# Autodesk Inventor assembly: CyberOrto
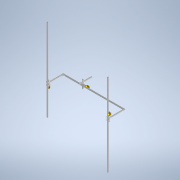
[picture p0: Inventor's stored thumbnail of the model, 180x180]
Saved by Autodesk Inventor 2022 (Build 260153000, 153)
## iProperties
RuleStatus: InUse
Created: 2021-12-29
Part Number: CyberOrto
Document SubType Name: Assembly
Designer: matte
Author: matte
## Documents named in this file (29)
- C:\Users\matte\Documents\GitHub\MDM-CyberOrto-CAD\CyberOrto.iam
- C:\Users\matte\Documents\GitHub\MDM-CyberOrto-CAD\Pezzi singoli\Trave Principale.ipt
- C:\Users\matte\Documents\GitHub\MDM-CyberOrto-CAD\Pezzi singoli\Supporto SX.ipt
- C:\Users\matte\Documents\GitHub\MDM-CyberOrto-CAD\Parker components\03-Brackets_Gussets_Plates\09-Machined Gussets\20-102.ipt
- C:\Users\matte\Documents\GitHub\MDM-CyberOrto-CAD\Parker components\02-Fasteners\10-Standard T-Nuts\20-050.ipt
- C:\Users\matte\Documents\GitHub\MDM-CyberOrto-CAD\Parker components\02-Fasteners\16-Screws\01-Metric Screws\01-Button Head\24-118-8.ipt
- C:\Users\matte\Documents\GitHub\MDM-CyberOrto-CAD\Guida a terra.iam
- C:\Users\matte\Documents\GitHub\MDM-CyberOrto-CAD\Parker components\05-Handles_Hinges\13-Pivot Joints\23-010.iam
- C:\Users\matte\Documents\GitHub\MDM-CyberOrto-CAD\Parker components\02-Fasteners\10-Standard T-Nuts\20-058.ipt
- C:\Users\matte\Documents\GitHub\MDM-CyberOrto-CAD\Parker components\02-Fasteners\16-Screws\01-Metric Screws\01-Button Head\24-116-8.ipt
- C:\Users\matte\Documents\GitHub\MDM-CyberOrto-CAD\Pezzi singoli\Supporto DX.ipt
- C:\Users\matte\Documents\GitHub\MDM-CyberOrto-CAD\Parker components\02-Fasteners\16-Screws\01-Metric Screws\01-Button Head\24-120-8.ipt
- C:\Users\matte\Documents\GitHub\MDM-CyberOrto-CAD\Pezzi singoli\Supporto lineare\Carrello semplice.iam
- C:\Users\matte\Documents\GitHub\MDM-CyberOrto-CAD\Platform.ipt
- C:\Users\matte\Documents\GitHub\MDM-CyberOrto-CAD\Parker components\02-Fasteners\16-Screws\01-Metric Screws\01-Button Head\24-130-6.ipt
- C:\Users\matte\Documents\GitHub\MDM-CyberOrto-CAD\Parker components\02-Fasteners\15-T-Bolts_Nuts_Washers\03-Washers\24-700-6.ipt
- C:\Users\matte\Documents\GitHub\MDM-CyberOrto-CAD\Parker components\02-Fasteners\15-T-Bolts_Nuts_Washers\02-Nuts\24-706-6.ipt
- C:\Users\matte\Documents\GitHub\MDM-CyberOrto-CAD\Servo Motor 50W\bch2mba531ca5c.ipt
- C:\Users\matte\Documents\GitHub\MDM-CyberOrto-CAD\Rack_Pinion\Rack gear scaled1.ipt
- C:\Users\matte\Documents\GitHub\MDM-CyberOrto-CAD\Rack_Pinion\pinion_scaled1.ipt
- C:\Users\matte\Documents\GitHub\MDM-CyberOrto-CAD\Inventor Support\Content Center Files\it-IT\ISO 1580\ISO 1580 - M4 x 12_.ipt
- C:\Users\matte\Documents\GitHub\MDM-CyberOrto-CAD\Inventor Support\Content Center Files\it-IT\AS 1474(1)\AS 1474 - M4(1).ipt
- C:\Users\matte\Documents\GitHub\MDM-CyberOrto-CAD\Trave a terra\Trave a terra.iam
- C:\Users\matte\Documents\GitHub\MDM-CyberOrto-CAD\Racks.iam
- C:\Users\matte\Documents\GitHub\MDM-CyberOrto-CAD\Parker components\02-Fasteners\16-Screws\01-Metric Screws\03-Socket Head\24-320-8SS.ipt
- C:\Users\matte\Documents\GitHub\MDM-CyberOrto-CAD\Parker components\02-Fasteners\10-Standard T-Nuts\20-058SS.ipt
- C:\Users\matte\Documents\GitHub\MDM-CyberOrto-CAD\Torretta.iam
- C:\Users\matte\Documents\GitHub\MDM-CyberOrto-CAD\Pezzi singoli\13-106_f.ipt
- C:\Users\matte\Documents\GitHub\MDM-CyberOrto-CAD\Pezzi singoli\13-513.ipt
## Components (129 placed, 28 different names)
1. Trave Principale:1 — Coincidente:1, Coincidente:2, Coincidente:3, Allineato:1, Coincidente:4, Allineato:2, Coincidente:5, Coincidente:10, Coincidente:40, Allineato:5, Allineato:6, Coincidente:41, Angolo:1, Angolo:7, Allineato:119, Coincidente:238, Allineato:120, Coincidente:239, Coincidente:245, Coincidente:257, Angolo:9, Allineato:141, Coincidente:259, Coincidente:260, Allineato:142, Coincidente:261, Coincidente:262, Allineato:143, Allineato:144, Coincidente:265
2. Supporto SX:1 — Allineato:1, Coincidente:4, Allineato:2, Coincidente:6, Allineato:3, Coincidente:7, Coincidente:15, Coincidente:16, Coincidente:23, Coincidente:28, Coincidente:29, Coincidente:30
3. Supporto DX:1 — Coincidente:45, Allineato:7, Allineato:8, Coincidente:48, Allineato:9, Allineato:10
4. Torretta:1 [sub-assembly] — Angolo:7, Coincidente:258, Coincidente:265, Allineato:145
5. pinion_scaled1:3 — Coincidente:258, Allineato:146
6. 13-106_f:1 — Allineato:142, Coincidente:261, Coincidente:262, Coincidente:264, Allineato:145
7. 13-106_f:2 — Allineato:141, Coincidente:259, Coincidente:260, Coincidente:263
8. 13-513:1 — Allineato:143, Coincidente:264
9. 13-513:2 — Allineato:144, Coincidente:263
10. 24-118-8:3 — Coincidente:19, Coincidente:20
11. 24-118-8:4 — Coincidente:21, Coincidente:22
12. 20-050:2 — Coincidente:10, Coincidente:11, Coincidente:12
13. 24-118-8:1 — Coincidente:13, Coincidente:14
14. 24-118-8:2 — Coincidente:17, Coincidente:18
15. 20-102:1 — Coincidente:5, Coincidente:6, Allineato:3, Coincidente:8, Coincidente:9, Coincidente:11, Coincidente:12, Coincidente:13, Coincidente:14, Coincidente:17, Coincidente:18, Coincidente:19, Coincidente:20, Coincidente:21, Coincidente:22
16. 20-050:1 — Coincidente:7, Coincidente:8, Coincidente:9
17. 24-118-8:5 — Coincidente:31, Coincidente:32, Coincidente:33
18. 24-118-8:6 — Coincidente:34, Coincidente:35
19. 24-118-8:7 — Coincidente:38, Coincidente:39
20. 24-118-8:8 — Coincidente:36, Coincidente:37
21. Guida a terra:1 [sub-assembly] — Coincidente:15, Coincidente:16, Coincidente:23, Coincidente:32, Coincidente:33, Coincidente:34, Coincidente:35, Coincidente:36, Coincidente:37, Coincidente:38, Coincidente:39, Coincidente:138, Coincidente:139, Allineato:61, Coincidente:141, Coincidente:143, Coincidente:145, Coincidente:162, Coincidente:210, Allineato:115
22. 20-050:3 — Coincidente:27, Allineato:4, Coincidente:28, Coincidente:30, Coincidente:31
23. 20-050:4 — Coincidente:27, Allineato:4, Coincidente:29
24. 23-010:1 [sub-assembly] — Coincidente:40, Allineato:5, Allineato:6, Coincidente:43, Coincidente:44, Coincidente:45, Allineato:7, Allineato:8, Coincidente:46, Coincidente:47
25. 20-058:1 — Coincidente:41, Angolo:1, Coincidente:42
26. 24-116-8:1 — Coincidente:42, Coincidente:43, Coincidente:44
27. 24-120-8:1 — Coincidente:46, Coincidente:47
28. 24-120-8:2 — Coincidente:51, Coincidente:52
29. Carrello semplice:1 [sub-assembly] — Coincidente:48, Allineato:9, Allineato:10, Coincidente:51, Coincidente:52, Coincidente:53, Allineato:13, Coincidente:54, Coincidente:56, Coincidente:58, Coincidente:60, Coincidente:62, Angolo:2, Angolo:3, Angolo:4, Allineato:59, Coincidente:130
30. 24-130-6:1 — Inserimento:1, Coincidente:61
31. 24-700-6:1 — Inserimento:1, Inserimento:7
32. 24-706-6:1 — Coincidente:55, Coincidente:56
33. 24-130-6:2 — Coincidente:59
34. 24-700-6:3 — Inserimento:6
35. 24-130-6:3 — Coincidente:57
36. 24-700-6:2 — Inserimento:8
37. 24-130-6:4 — Coincidente:55
38. 24-700-6:4 — Inserimento:5
39. 24-706-6:2 — Coincidente:57, Coincidente:58
40. 24-706-6:3 — Coincidente:61, Coincidente:62
41. 24-706-6:4 — Coincidente:59, Coincidente:60
42. Platform:1 — Coincidente:53, Allineato:13, Coincidente:54, Inserimento:5, Inserimento:6, Inserimento:7, Inserimento:8, Coincidente:66, Coincidente:67, Coincidente:68, Coincidente:114, Coincidente:117, Coincidente:121, Coincidente:125, Coincidente:129
43. ISO 1580 M4 x 12:2 — Coincidente:126, Coincidente:127, Coincidente:128
44. AS 1474 - Metrico M4:2 — Coincidente:120, Coincidente:121
45. AS 1474 - Metrico M4:3 — Coincidente:124, Coincidente:125
46. AS 1474 - Metrico M4:4 — Coincidente:128, Coincidente:129
47. ISO 1580 M4 x 12:4 — Coincidente:118, Coincidente:119, Coincidente:120
48. ISO 1580 M4 x 12:3 — Coincidente:122, Coincidente:123, Coincidente:124
49. AS 1474 - Metrico M4:1 — Coincidente:116, Coincidente:117
50. ISO 1580 M4 x 12:1 — Coincidente:114, Coincidente:115, Coincidente:116
51. bch2mba531ca5c:1 — Coincidente:66, Coincidente:67, Coincidente:68, Coincidente:113, Coincidente:115, Coincidente:118, Coincidente:119, Coincidente:122, Coincidente:123, Coincidente:126, Coincidente:127
52. 24-706-6:8 — Coincidente:142, Coincidente:143
53. 24-706-6:7 — Coincidente:140, Coincidente:141
54. 24-706-6:6 — Coincidente:144, Coincidente:145
55. 24-700-6:8
56. 24-130-6:8 — Coincidente:146
57. 24-700-6:7
58. 24-130-6:7 — Coincidente:144
59. 24-700-6:6
60. 24-706-6:5 — Coincidente:146, Coincidente:162
61. 24-700-6:5
62. Platform:3 — Coincidente:138, Coincidente:139, Allineato:61, Coincidente:158, Coincidente:159, Coincidente:160, Coincidente:164, Coincidente:166, Coincidente:167, Coincidente:168
63. 24-130-6:5 — Coincidente:142
64. 24-130-6:6 — Coincidente:140
65. bch2mba531ca5c:2 — Coincidente:158, Coincidente:161, Coincidente:211
66. ISO 1580 M4 x 12:5 — Coincidente:161
67. AS 1474 - Metrico M4:5 — Coincidente:167
68. ISO 1580 M4 x 12:6 — Coincidente:159, Coincidente:163
69. AS 1474 - Metrico M4:6 — Coincidente:168
70. AS 1474 - Metrico M4:7 — Coincidente:165, Coincidente:166
71. ISO 1580 M4 x 12:7 — Coincidente:165
72. AS 1474 - Metrico M4:8 — Coincidente:163, Coincidente:164
73. ISO 1580 M4 x 12:8 — Coincidente:160
74. pinion_scaled1:1 — Coincidente:113, Allineato:87
75. Trave a terra:1 [sub-assembly] — Angolo:2, Angolo:3, Angolo:4, Allineato:59, Coincidente:130, Coincidente:169, Angolo:5, Coincidente:171, Allineato:62, Allineato:88, Coincidente:187, Coincidente:189
76. 20-058SS:2 — Coincidente:188, Coincidente:189
77. 20-058SS:1 — Coincidente:186, Coincidente:187
78. Racks:5 [sub-assembly] — Allineato:73, Allineato:74, Coincidente:177, Allineato:75, Allineato:76, Coincidente:178
79. Racks:6 [sub-assembly] — Allineato:75, Allineato:76, Coincidente:178, Coincidente:180, Allineato:77, Allineato:78
80. Racks:7 [sub-assembly] — Coincidente:180, Allineato:77, Allineato:78, Allineato:79, Allineato:80, Coincidente:181
81. Racks:8 [sub-assembly] — Allineato:79, Allineato:80, Coincidente:181, Coincidente:182, Allineato:81, Allineato:82
82. Racks:9 [sub-assembly] — Coincidente:182, Allineato:81, Allineato:82, Allineato:85, Allineato:86, Coincidente:185
83. Rack gear scaled1:2 — Allineato:85, Allineato:86, Coincidente:185
84. 24-320-8SS:3
85. 24-320-8SS:4 — Coincidente:188
86. Racks:4 [sub-assembly] — Coincidente:174, Allineato:67, Allineato:68, Allineato:69, Allineato:70, Coincidente:175
87. Racks:3 [sub-assembly] — Allineato:71, Coincidente:176, Allineato:72, Allineato:73, Allineato:74, Coincidente:177
88. Racks:2 [sub-assembly] — Allineato:69, Allineato:70, Coincidente:175, Allineato:71, Coincidente:176, Allineato:72
89. Rack gear scaled1:1 — Coincidente:170, Coincidente:171, Allineato:62, Allineato:63, Allineato:64, Coincidente:172, Allineato:65, Coincidente:173, Allineato:66
90. 24-320-8SS:1 — Coincidente:172, Allineato:65, Coincidente:186
91. 24-320-8SS:2 — Coincidente:173, Allineato:66
92. Racks:1 [sub-assembly] — Coincidente:169, Angolo:5, Coincidente:170, Allineato:63, Allineato:64, Coincidente:174, Allineato:67, Allineato:68, Allineato:87, Allineato:88
93. pinion_scaled1:2 — Coincidente:211, Allineato:116
94. Trave a terra:2 [sub-assembly] — Coincidente:210, Allineato:115
95. 20-058SS:4
96. 24-320-8SS:8
97. 24-320-8SS:7
98. Rack gear scaled1:4
99. Racks:18 [sub-assembly]
100. Racks:17 [sub-assembly]
101. Racks:16 [sub-assembly]
102. Racks:15 [sub-assembly]
103. Racks:14 [sub-assembly]
104. Racks:11 [sub-assembly] — Allineato:116
105. Racks:12 [sub-assembly]
106. Racks:13 [sub-assembly]
107. Racks:10 [sub-assembly]
108. Rack gear scaled1:3
109. 24-320-8SS:5
110. 24-320-8SS:6
111. 20-058SS:3
112. Rack gear scaled1:5 — Allineato:119, Coincidente:238, Allineato:120, Angolo:8, Coincidente:246, Allineato:131
113. 24-320-8SS:9
114. 24-320-8SS:10
115. 20-058SS:5 — Angolo:8, Coincidente:239
116. Racks:19 [sub-assembly] — Coincidente:250, Allineato:139, Allineato:140
117. Racks:20 [sub-assembly]
118. Racks:21 [sub-assembly] — Coincidente:245
119. Racks:22 [sub-assembly]
120. Racks:23 [sub-assembly] — Allineato:146
121. Racks:24 [sub-assembly] — Coincidente:246, Allineato:131
122. Rack gear scaled1:6 — Coincidente:250, Allineato:134, Allineato:137, Coincidente:255, Allineato:138, Allineato:139, Allineato:140
123. 24-320-8SS:11 — Coincidente:251
124. 24-320-8SS:12
125. 20-050:5 — Coincidente:251, Allineato:134, Coincidente:254
126. Rack gear scaled1:7 — Allineato:137, Coincidente:255, Allineato:138
127. 24-320-8SS:14 — Coincidente:254
128. 24-320-8SS:13 — Coincidente:256
129. 20-058SS:6 — Coincidente:256, Coincidente:257, Angolo:9
## Relationships (302: Mate 179, Flush 98, Insert 16, Angle 9)
- Coincidente:1 [Mate]: Trave Principale:1
- Coincidente:2 [Mate]: Trave Principale:1
- Coincidente:3 [Mate]: Trave Principale:1
- Allineato:1 [Flush]: Trave Principale:1 ↔ Supporto SX:1
- Coincidente:4 [Mate]: Trave Principale:1 ↔ Supporto SX:1
- Allineato:2 [Flush]: Trave Principale:1 ↔ Supporto SX:1
- Coincidente:5 [Mate]: Trave Principale:1 ↔ 20-102:1
- Coincidente:6 [Mate]: Supporto SX:1 ↔ 20-102:1
- Allineato:3 [Flush]: Supporto SX:1 ↔ 20-102:1
- Coincidente:7 [Mate]: Supporto SX:1 ↔ 20-050:1
- Coincidente:8 [Mate]: 20-102:1 ↔ 20-050:1
- Coincidente:9 [Mate]: 20-102:1 ↔ 20-050:1
- Coincidente:10 [Mate]: Trave Principale:1 ↔ 20-050:2
- Coincidente:11 [Mate]: 20-050:2 ↔ 20-102:1
- Coincidente:12 [Mate]: 20-050:2 ↔ 20-102:1
- Coincidente:13 [Mate]: 24-118-8:1 ↔ 20-102:1
- Coincidente:14 [Mate]: 24-118-8:1 ↔ 20-102:1
- Coincidente:15 [Mate]: Supporto SX:1 ↔ Guida a terra:1
- Coincidente:16 [Mate]: Supporto SX:1 ↔ Guida a terra:1
- Coincidente:17 [Mate]: 24-118-8:2 ↔ 20-102:1
- Coincidente:18 [Mate]: 24-118-8:2 ↔ 20-102:1
- Coincidente:19 [Mate]: 24-118-8:3 ↔ 20-102:1
- Coincidente:20 [Mate]: 24-118-8:3 ↔ 20-102:1
- Coincidente:21 [Mate]: 24-118-8:4 ↔ 20-102:1
- Coincidente:22 [Mate]: 24-118-8:4 ↔ 20-102:1
- Coincidente:23 [Mate]: Supporto SX:1 ↔ Guida a terra:1
- Coincidente:27 [Mate]: 20-050:3 ↔ 20-050:4
- Allineato:4 [Flush]: 20-050:3 ↔ 20-050:4
- Coincidente:28 [Mate]: Supporto SX:1 ↔ 20-050:3
- Coincidente:29 [Mate]: Supporto SX:1 ↔ 20-050:4
- Coincidente:30 [Mate]: Supporto SX:1 ↔ 20-050:3
- Coincidente:31 [Mate]: 24-118-8:5 ↔ 20-050:3
- Coincidente:32 [Mate]: 24-118-8:5 ↔ Guida a terra:1
- Coincidente:33 [Mate]: 24-118-8:5 ↔ Guida a terra:1
- Coincidente:34 [Mate]: 24-118-8:6 ↔ Guida a terra:1
- Coincidente:35 [Mate]: 24-118-8:6 ↔ Guida a terra:1
- Coincidente:36 [Mate]: 24-118-8:8 ↔ Guida a terra:1
- Coincidente:37 [Mate]: 24-118-8:8 ↔ Guida a terra:1
- Coincidente:38 [Mate]: 24-118-8:7 ↔ Guida a terra:1
- Coincidente:39 [Mate]: 24-118-8:7 ↔ Guida a terra:1
- Coincidente:40 [Mate]: Trave Principale:1 ↔ 23-010:1
- Allineato:5 [Flush]: Trave Principale:1 ↔ 23-010:1
- Allineato:6 [Flush]: Trave Principale:1 ↔ 23-010:1
- Coincidente:41 [Mate]: Trave Principale:1 ↔ 20-058:1
- Angolo:1 [Angle] (0 deg): Trave Principale:1 ↔ 20-058:1
- Coincidente:42 [Mate]: 20-058:1 ↔ 24-116-8:1
- Coincidente:43 [Mate]: 23-010:1 ↔ 24-116-8:1
- Coincidente:44 [Mate]: 23-010:1 ↔ 24-116-8:1
- Coincidente:45 [Mate]: Supporto DX:1 ↔ 23-010:1
- Allineato:7 [Flush]: Supporto DX:1 ↔ 23-010:1
- Allineato:8 [Flush]: Supporto DX:1 ↔ 23-010:1
- Coincidente:46 [Mate]: 23-010:1 ↔ 24-120-8:1
- Coincidente:47 [Mate]: 23-010:1 ↔ 24-120-8:1
- Coincidente:48 [Mate]: Supporto DX:1 ↔ Carrello semplice:1
- Allineato:9 [Flush]: Supporto DX:1 ↔ Carrello semplice:1
- Allineato:10 [Flush]: Supporto DX:1 ↔ Carrello semplice:1
- Coincidente:51 [Mate]: 24-120-8:2 ↔ Carrello semplice:1
- Coincidente:52 [Mate]: 24-120-8:2 ↔ Carrello semplice:1
- Coincidente:53 [Mate]: Carrello semplice:1 ↔ Platform:1
- Allineato:13 [Flush]: Carrello semplice:1 ↔ Platform:1
- Coincidente:54 [Mate]: Carrello semplice:1 ↔ Platform:1
- Inserimento:1: 24-130-6:1 ↔ 24-700-6:1
- [Insert]: 24-130-6:2 ↔ 24-700-6:2
- [Insert]: 24-700-6:3 ↔ 24-130-6:3
- [Insert]: 24-130-6:4 ↔ 24-700-6:4
- Inserimento:5: 24-700-6:4 ↔ Platform:1
- Inserimento:6: 24-700-6:3 ↔ Platform:1
- Inserimento:7: 24-700-6:1 ↔ Platform:1
- Inserimento:8: 24-700-6:2 ↔ Platform:1
- Coincidente:55 [Mate]: 24-706-6:1 ↔ 24-130-6:4
- Coincidente:56 [Mate]: Carrello semplice:1 ↔ 24-706-6:1
- Coincidente:57 [Mate]: 24-130-6:3 ↔ 24-706-6:2
- Coincidente:58 [Mate]: Carrello semplice:1 ↔ 24-706-6:2
- Coincidente:59 [Mate]: 24-130-6:2 ↔ 24-706-6:4
- Coincidente:60 [Mate]: Carrello semplice:1 ↔ 24-706-6:4
- Coincidente:61 [Mate]: 24-130-6:1 ↔ 24-706-6:3
- Coincidente:62 [Mate]: Carrello semplice:1 ↔ 24-706-6:3
- Coincidente:66 [Mate]: Platform:1 ↔ bch2mba531ca5c:1
- Coincidente:67 [Mate]: Platform:1 ↔ bch2mba531ca5c:1
- Coincidente:68 [Mate]: Platform:1 ↔ bch2mba531ca5c:1
- Coincidente:113 [Mate]: bch2mba531ca5c:1 ↔ pinion_scaled1:1
- Coincidente:114 [Mate]: Platform:1 ↔ ISO 1580 M4 x 12:1
- Coincidente:115 [Mate]: ISO 1580 M4 x 12:1 ↔ bch2mba531ca5c:1
- Coincidente:116 [Mate]: AS 1474 - Metrico M4:1 ↔ ISO 1580 M4 x 12:1
- Coincidente:117 [Mate]: Platform:1 ↔ AS 1474 - Metrico M4:1
- Coincidente:118 [Mate]: ISO 1580 M4 x 12:4 ↔ bch2mba531ca5c:1
- Coincidente:119 [Mate]: ISO 1580 M4 x 12:4 ↔ bch2mba531ca5c:1
- Coincidente:120 [Mate]: AS 1474 - Metrico M4:2 ↔ ISO 1580 M4 x 12:4
- Coincidente:121 [Mate]: Platform:1 ↔ AS 1474 - Metrico M4:2
- Coincidente:122 [Mate]: ISO 1580 M4 x 12:3 ↔ bch2mba531ca5c:1
- Coincidente:123 [Mate]: ISO 1580 M4 x 12:3 ↔ bch2mba531ca5c:1
- Coincidente:124 [Mate]: AS 1474 - Metrico M4:3 ↔ ISO 1580 M4 x 12:3
- Coincidente:125 [Mate]: Platform:1 ↔ AS 1474 - Metrico M4:3
- Coincidente:126 [Mate]: ISO 1580 M4 x 12:2 ↔ bch2mba531ca5c:1
- Coincidente:127 [Mate]: ISO 1580 M4 x 12:2 ↔ bch2mba531ca5c:1
- Coincidente:128 [Mate]: ISO 1580 M4 x 12:2 ↔ AS 1474 - Metrico M4:4
- Coincidente:129 [Mate]: Platform:1 ↔ AS 1474 - Metrico M4:4
- Angolo:2 [Angle] (0 deg): Carrello semplice:1 ↔ Trave a terra:1
- Angolo:3 [Angle] (0 deg): Carrello semplice:1 ↔ Trave a terra:1
- Angolo:4 [Angle] (0 deg): Carrello semplice:1 ↔ Trave a terra:1
- Allineato:59 [Flush] (19 mm): Carrello semplice:1 ↔ Trave a terra:1
- Coincidente:130 [Mate] (20 mm): Carrello semplice:1 ↔ Trave a terra:1
- [Insert]: 24-700-6:5 ↔ 24-130-6:5
- [Insert]: 24-700-6:6 ↔ 24-130-6:6
- [Insert]: 24-700-6:7 ↔ 24-130-6:7
- [Insert]: 24-700-6:8 ↔ 24-130-6:8
- [Insert]: 24-700-6:8 ↔ Platform:3
- [Insert]: 24-700-6:7 ↔ Platform:3
- [Insert]: 24-700-6:5 ↔ Platform:3
- [Insert]: 24-700-6:6 ↔ Platform:3
- Coincidente:138 [Mate]: Guida a terra:1 ↔ Platform:3
- Coincidente:139 [Mate]: Guida a terra:1 ↔ Platform:3
- Allineato:61 [Flush]: Guida a terra:1 ↔ Platform:3
- Coincidente:140 [Mate]: 24-706-6:7 ↔ 24-130-6:6
- Coincidente:141 [Mate]: Guida a terra:1 ↔ 24-706-6:7
- Coincidente:142 [Mate]: 24-706-6:8 ↔ 24-130-6:5
- Coincidente:143 [Mate]: Guida a terra:1 ↔ 24-706-6:8
- Coincidente:144 [Mate]: 24-706-6:6 ↔ 24-130-6:7
- Coincidente:145 [Mate]: Guida a terra:1 ↔ 24-706-6:6
- Coincidente:146 [Mate]: 24-130-6:8 ↔ 24-706-6:5
- [Mate]: bch2mba531ca5c:2 ↔ ISO 1580 M4 x 12:5
- [Mate]: ISO 1580 M4 x 12:5 ↔ AS 1474 - Metrico M4:5
- [Mate]: bch2mba531ca5c:2 ↔ ISO 1580 M4 x 12:8
- [Mate]: bch2mba531ca5c:2 ↔ ISO 1580 M4 x 12:8
- [Mate]: AS 1474 - Metrico M4:6 ↔ ISO 1580 M4 x 12:8
- [Mate]: bch2mba531ca5c:2 ↔ ISO 1580 M4 x 12:7
- [Mate]: bch2mba531ca5c:2 ↔ ISO 1580 M4 x 12:7
- [Mate]: bch2mba531ca5c:2 ↔ ISO 1580 M4 x 12:6
- [Mate]: bch2mba531ca5c:2 ↔ ISO 1580 M4 x 12:6
- Coincidente:158 [Mate]: Platform:3 ↔ bch2mba531ca5c:2
- Coincidente:159 [Mate]: Platform:3 ↔ ISO 1580 M4 x 12:6
- Coincidente:160 [Mate]: Platform:3 ↔ ISO 1580 M4 x 12:8
- Coincidente:161 [Mate]: bch2mba531ca5c:2 ↔ ISO 1580 M4 x 12:5
- Coincidente:162 [Mate]: Guida a terra:1 ↔ 24-706-6:5
- Coincidente:163 [Mate]: ISO 1580 M4 x 12:6 ↔ AS 1474 - Metrico M4:8
- Coincidente:164 [Mate]: Platform:3 ↔ AS 1474 - Metrico M4:8
- Coincidente:165 [Mate]: AS 1474 - Metrico M4:7 ↔ ISO 1580 M4 x 12:7
- Coincidente:166 [Mate]: Platform:3 ↔ AS 1474 - Metrico M4:7
- Coincidente:167 [Mate]: Platform:3 ↔ AS 1474 - Metrico M4:5
- Coincidente:168 [Mate]: Platform:3 ↔ AS 1474 - Metrico M4:6
- Coincidente:169 [Mate]: Trave a terra:1 ↔ Racks:1
- Angolo:5 [Angle] (0 deg): Trave a terra:1 ↔ Racks:1
- Coincidente:170 [Mate]: Rack gear scaled1:1 ↔ Racks:1
- Coincidente:171 [Mate]: Trave a terra:1 ↔ Rack gear scaled1:1
- Allineato:62 [Flush]: Trave a terra:1 ↔ Rack gear scaled1:1
- Allineato:63 [Flush]: Rack gear scaled1:1 ↔ Racks:1
- Allineato:64 [Flush]: Rack gear scaled1:1 ↔ Racks:1
- Coincidente:172 [Mate]: Rack gear scaled1:1 ↔ 24-320-8SS:1
- Allineato:65 [Flush]: Rack gear scaled1:1 ↔ 24-320-8SS:1
- Coincidente:173 [Mate]: Rack gear scaled1:1 ↔ 24-320-8SS:2
- Allineato:66 [Flush]: Rack gear scaled1:1 ↔ 24-320-8SS:2
- Coincidente:174 [Mate]: Racks:4 ↔ Racks:1
- Allineato:67 [Flush]: Racks:4 ↔ Racks:1
- Allineato:68 [Flush]: Racks:4 ↔ Racks:1
- Allineato:69 [Flush]: Racks:4 ↔ Racks:2
- Allineato:70 [Flush]: Racks:4 ↔ Racks:2
- Coincidente:175 [Mate]: Racks:4 ↔ Racks:2
- Allineato:71 [Flush]: Racks:3 ↔ Racks:2
- Coincidente:176 [Mate]: Racks:3 ↔ Racks:2
- Allineato:72 [Flush]: Racks:3 ↔ Racks:2
- Allineato:73 [Flush]: Racks:5 ↔ Racks:3
- Allineato:74 [Flush]: Racks:5 ↔ Racks:3
- Coincidente:177 [Mate]: Racks:5 ↔ Racks:3
- Allineato:75 [Flush]: Racks:5 ↔ Racks:6
- Allineato:76 [Flush]: Racks:5 ↔ Racks:6
- Coincidente:178 [Mate]: Racks:5 ↔ Racks:6
- Coincidente:180 [Mate]: Racks:6 ↔ Racks:7
- Allineato:77 [Flush]: Racks:6 ↔ Racks:7
- Allineato:78 [Flush]: Racks:6 ↔ Racks:7
- Allineato:79 [Flush]: Racks:7 ↔ Racks:8
- Allineato:80 [Flush]: Racks:7 ↔ Racks:8
- Coincidente:181 [Mate]: Racks:7 ↔ Racks:8
- Coincidente:182 [Mate]: Racks:8 ↔ Racks:9
- Allineato:81 [Flush]: Racks:8 ↔ Racks:9
- Allineato:82 [Flush]: Racks:8 ↔ Racks:9
- [Mate]: Rack gear scaled1:2 ↔ 24-320-8SS:3
- [Flush]: Rack gear scaled1:2 ↔ 24-320-8SS:3
- [Mate]: Rack gear scaled1:2 ↔ 24-320-8SS:4
- [Flush]: Rack gear scaled1:2 ↔ 24-320-8SS:4
- Allineato:85 [Flush]: Racks:9 ↔ Rack gear scaled1:2
- Allineato:86 [Flush]: Racks:9 ↔ Rack gear scaled1:2
- Coincidente:185 [Mate]: Racks:9 ↔ Rack gear scaled1:2
- Allineato:87 [Flush]: pinion_scaled1:1 ↔ Racks:1
- Allineato:88 [Flush] (-13 mm): Trave a terra:1 ↔ Racks:1
- Coincidente:186 [Mate]: 20-058SS:1 ↔ 24-320-8SS:1
- Coincidente:187 [Mate]: Trave a terra:1 ↔ 20-058SS:1
- Coincidente:188 [Mate]: 20-058SS:2 ↔ 24-320-8SS:4
- Coincidente:189 [Mate]: Trave a terra:1 ↔ 20-058SS:2
- [Mate]: Trave a terra:2 ↔ Racks:10
- [Angle] (0 deg): Trave a terra:2 ↔ Racks:10
- [Mate]: Racks:10 ↔ Rack gear scaled1:3
- [Mate]: Trave a terra:2 ↔ Rack gear scaled1:3
- [Flush]: Trave a terra:2 ↔ Rack gear scaled1:3
- [Flush]: Racks:10 ↔ Rack gear scaled1:3
- [Flush]: Racks:10 ↔ Rack gear scaled1:3
- [Mate]: Rack gear scaled1:3 ↔ 24-320-8SS:5
- [Flush]: Rack gear scaled1:3 ↔ 24-320-8SS:5
- [Mate]: Rack gear scaled1:3 ↔ 24-320-8SS:6
- [Flush]: Rack gear scaled1:3 ↔ 24-320-8SS:6
- [Mate]: Racks:13 ↔ Racks:10
- [Flush]: Racks:13 ↔ Racks:10
- [Flush]: Racks:13 ↔ Racks:10
- [Flush]: Racks:11 ↔ Racks:13
- [Flush]: Racks:11 ↔ Racks:13
- [Mate]: Racks:11 ↔ Racks:13
- [Flush]: Racks:11 ↔ Racks:12
- [Mate]: Racks:11 ↔ Racks:12
- [Flush]: Racks:11 ↔ Racks:12
- [Flush]: Racks:14 ↔ Racks:12
- [Flush]: Racks:14 ↔ Racks:12
- [Mate]: Racks:14 ↔ Racks:12
- [Flush]: Racks:15 ↔ Racks:14
- [Flush]: Racks:15 ↔ Racks:14
- [Mate]: Racks:15 ↔ Racks:14
- [Mate]: Racks:16 ↔ Racks:15
- [Flush]: Racks:16 ↔ Racks:15
- [Flush]: Racks:16 ↔ Racks:15
- [Flush]: Racks:17 ↔ Racks:16
- [Flush]: Racks:17 ↔ Racks:16
- [Mate]: Racks:17 ↔ Racks:16
- [Mate]: Racks:18 ↔ Racks:17
- [Flush]: Racks:18 ↔ Racks:17
- [Flush]: Racks:18 ↔ Racks:17
- [Mate]: 24-320-8SS:7 ↔ Rack gear scaled1:4
- [Flush]: 24-320-8SS:7 ↔ Rack gear scaled1:4
- [Mate]: 24-320-8SS:8 ↔ Rack gear scaled1:4
- [Flush]: 24-320-8SS:8 ↔ Rack gear scaled1:4
- [Flush]: Rack gear scaled1:4 ↔ Racks:18
- [Flush]: Rack gear scaled1:4 ↔ Racks:18
- [Mate]: Rack gear scaled1:4 ↔ Racks:18
- [Flush] (-13 mm): Trave a terra:2 ↔ Racks:10
- [Mate]: 24-320-8SS:5 ↔ 20-058SS:3
- [Mate]: Trave a terra:2 ↔ 20-058SS:3
- [Mate]: 20-058SS:4 ↔ 24-320-8SS:8
- [Mate]: Trave a terra:2 ↔ 20-058SS:4
- Coincidente:210 [Mate] (20 mm): Guida a terra:1 ↔ Trave a terra:2
- Allineato:115 [Flush] (19 mm): Guida a terra:1 ↔ Trave a terra:2
- Coincidente:211 [Mate]: bch2mba531ca5c:2 ↔ pinion_scaled1:2
- Allineato:116 [Flush]: pinion_scaled1:2 ↔ Racks:11
- Angolo:7 [Angle] (180 deg): Trave Principale:1 ↔ Torretta:1
- [Mate]: Rack gear scaled1:5 ↔ 24-320-8SS:9
- [Flush]: Rack gear scaled1:5 ↔ 24-320-8SS:9
- [Mate]: Rack gear scaled1:5 ↔ 24-320-8SS:10
- [Flush]: Rack gear scaled1:5 ↔ 24-320-8SS:10
- [Mate]: 24-320-8SS:10 ↔ 20-058SS:5
- Allineato:119 [Flush]: Trave Principale:1 ↔ Rack gear scaled1:5
- Coincidente:238 [Mate]: Trave Principale:1 ↔ Rack gear scaled1:5
- Allineato:120 [Flush] (13 mm): Trave Principale:1 ↔ Rack gear scaled1:5
- Angolo:8 [Angle] (0 deg): Rack gear scaled1:5 ↔ 20-058SS:5
- Coincidente:239 [Mate]: Trave Principale:1 ↔ 20-058SS:5
- [Mate]: Racks:19 ↔ Racks:22
- [Flush]: Racks:19 ↔ Racks:22
- [Flush]: Racks:19 ↔ Racks:22
- [Flush]: Racks:20 ↔ Racks:22
- [Flush]: Racks:20 ↔ Racks:22
- [Mate]: Racks:20 ↔ Racks:22
- [Flush]: Racks:20 ↔ Racks:21
- [Mate]: Racks:20 ↔ Racks:21
- [Flush]: Racks:20 ↔ Racks:21
- [Flush]: Racks:21 ↔ Racks:23
- [Flush]: Racks:21 ↔ Racks:23
- [Mate]: Racks:21 ↔ Racks:23
- [Flush]: Racks:23 ↔ Racks:24
- [Flush]: Racks:23 ↔ Racks:24
- [Mate]: Racks:23 ↔ Racks:24
- Coincidente:245 [Mate]: Trave Principale:1 ↔ Racks:21
- Coincidente:246 [Mate]: Rack gear scaled1:5 ↔ Racks:24
- Allineato:131 [Flush]: Rack gear scaled1:5 ↔ Racks:24
- [Mate]: Rack gear scaled1:6 ↔ 24-320-8SS:11
- [Flush]: Rack gear scaled1:6 ↔ 24-320-8SS:11
- [Mate]: Rack gear scaled1:6 ↔ 24-320-8SS:12
- [Flush]: Rack gear scaled1:6 ↔ 24-320-8SS:12
- Coincidente:250 [Mate]: Racks:19 ↔ Rack gear scaled1:6
- Coincidente:251 [Mate]: 24-320-8SS:11 ↔ 20-050:5
- Allineato:134 [Flush] (-23.224 mm): Rack gear scaled1:6 ↔ 20-050:5
- [Mate]: Rack gear scaled1:7 ↔ 24-320-8SS:13
- [Flush]: Rack gear scaled1:7 ↔ 24-320-8SS:13
- [Mate]: Rack gear scaled1:7 ↔ 24-320-8SS:14
- [Flush]: Rack gear scaled1:7 ↔ 24-320-8SS:14
- Coincidente:254 [Mate]: 20-050:5 ↔ 24-320-8SS:14
- Allineato:137 [Flush]: Rack gear scaled1:6 ↔ Rack gear scaled1:7
- Coincidente:255 [Mate]: Rack gear scaled1:6 ↔ Rack gear scaled1:7
- Allineato:138 [Flush]: Rack gear scaled1:6 ↔ Rack gear scaled1:7
- Allineato:139 [Flush]: Racks:19 ↔ Rack gear scaled1:6
- Allineato:140 [Flush]: Racks:19 ↔ Rack gear scaled1:6
- Coincidente:256 [Mate]: 24-320-8SS:13 ↔ 20-058SS:6
- Coincidente:257 [Mate]: Trave Principale:1 ↔ 20-058SS:6
- Angolo:9 [Angle] (0 deg): Trave Principale:1 ↔ 20-058SS:6
- Coincidente:258 [Mate]: Torretta:1 ↔ pinion_scaled1:3
- Allineato:141 [Flush]: Trave Principale:1 ↔ 13-106_f:2
- Coincidente:259 [Mate]: Trave Principale:1 ↔ 13-106_f:2
- Coincidente:260 [Mate]: Trave Principale:1 ↔ 13-106_f:2
- Allineato:142 [Flush]: Trave Principale:1 ↔ 13-106_f:1
- Coincidente:261 [Mate]: Trave Principale:1 ↔ 13-106_f:1
- Coincidente:262 [Mate]: Trave Principale:1 ↔ 13-106_f:1
- Allineato:143 [Flush]: Trave Principale:1 ↔ 13-513:1
- Allineato:144 [Flush]: Trave Principale:1 ↔ 13-513:2
- Coincidente:263 [Mate]: 13-106_f:2 ↔ 13-513:2
- Coincidente:264 [Mate]: 13-106_f:1 ↔ 13-513:1
- Coincidente:265 [Mate] (20 mm): Trave Principale:1 ↔ Torretta:1
- Allineato:145 [Flush] (19 mm): Torretta:1 ↔ 13-106_f:1
- Allineato:146 [Flush]: pinion_scaled1:3 ↔ Racks:23
## Named parameters: L_piatto_guide = 240 mm, L_tracce_terra = 4000 mm, L_traccia_superiore = 3000 mm, H_supporto = 700 mm, d116_d115 = 0 mm, d117_d115 = 0 mm, d118_d115 = 0 mm, d311_d115 = 0 mm, d312_d116_d115 = 0 mm, d313_d117_d115 = 0 mm, d314_d118_d115 = 0 mm, d315_d119 = 0 mm, d316_d120 = 0 mm, d317_d121 = 0 mm, d318_d122 = 0 mm, d333_d234 = 0 mm, d334_d235 = 0 mm, d335_d237 = 0 mm, d336_d238 = 0 mm, d337_d239 = 0 mm, d338_d241 = 0 mm, d339_d242 = 0 mm, d341_d245 = 0 mm, d342_d246 = 0 mm, d398_d369 = 0 mm, d399_d370 = 0 mm, d400_d371 = 0 mm, d401_d372 = 0 mm, d411_d392 = 0 mm, d412_d393 = 0 mm, d413_d394 = 0 mm, d414_d395 = 0 mm, d415_d396 = 0 mm, d416_d397 = 0 mm, d417_d398_d369 = 0 mm, d418_d399_d370 = 0 mm, d419_d400_d371 = 0 mm, d420_d401_d372 = 0 mm, d421_d402 = 0 mm, d422_d403 = 0 mm, d423_d404 = 0 mm, d424_d406 = -13 mm, d425_d407 = 0 mm, d426_d408 = 0 mm, d427_d409 = 0 mm, d428_d410 = 0 mm, d429_d358 = 0 mm, d430_d359 = 0 deg, d431_d361 = 0 mm, d432_d362 = 0 mm, d433_d363 = 0 mm, d434_d364 = 0 mm, d435_d365 = 0 mm, d436_d369 = 0 mm, d437_d370 = 0 mm, d438_d371 = 0 mm, d439_d372 = 0 mm, d440_d373 = 0 mm, d441_d374 = 0 mm, d442_d375 = 0 mm, d443_d376 = 0 mm, d444_d377 = 0 mm, d445_d378 = 0 mm, d446_d379 = 0 mm, d447_d380 = 0 mm, d448_d381 = 0 mm, d449_d382 = 0 mm, d450_d383 = 0 mm, d451_d384 = 0 mm, d452_d385 = 0 mm, d453_d386 = 0 mm, d454_d387 = 0 mm, d455_d389 = 0 mm, d456_d390 = 0 mm, d457_d391 = 0 mm, d495_d398_d369 = 0 mm, d496_d399_d370 = 0 mm, d497_d400_d371 = 0 mm, d498_d401_d372 = 0 mm, d499_d409 = 0 mm, d511_d440_d373 = 0 mm, d512_d441_d374 = 0 mm, d513_d442_d375 = 0 mm, d514_d443_d376 = 0 mm, d515_d444_d377 = 0 mm, d516_d445_d378 = 0 mm, d517_d446_d379 = 0 mm, d518_d447_d380 = 0 mm, d519_d448_d381 = 0 mm, d520_d449_d382 = 0 mm, d521_d450_d383 = 0 mm, d522_d451_d384 = 0 mm, d523_d452_d385 = 0 mm, d524_d453_d386 = 0 mm, d525_d454_d387 = 0 mm, d530_d495_d398_d369 = 0 mm, d531_d496_d399_d370 = 0 mm, d532_d497_d400_d371 = 0 mm, d533_d498_d401_d372 = 0 mm, d538_d530_d495_d398_d369 = 0 mm, d539_d531_d496_d399_d370 = 0 mm, d540_d532_d497_d400_d371 = 0 mm, d541_d533_d498_d401_d372 = 0 mm
